# Autodesk Inventor assembly: ENSAMBLAJE_VENTOSA_1
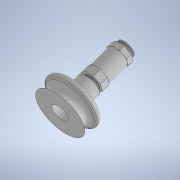
[picture p0: Inventor's stored thumbnail of the model, 180x180]
Saved by Autodesk Inventor 2022 (Build 260153000, 153)
## iProperties
Created: 2022-10-31
Part Number: ENSAMBLAJE_VENTOSA_1
Document SubType Name: Assembly
Designer: Usuario
Author: Usuario
## Documents named in this file (4)
- C:\Users\Usuario\Documents\Cosas de Sebastian\Robotica\PROYECTO\CAD\HERRAMIENTA\ENSAMBLAJE_VENTOSA_1.iam
- C:\Users\Usuario\Documents\Cosas de Sebastian\Robotica\PROYECTO\CAD\HERRAMIENTA\TORNILLO.ipt
- C:\Users\Usuario\Documents\Cosas de Sebastian\Robotica\PROYECTO\CAD\HERRAMIENTA\TUBO_METALICO.ipt
- C:\Users\Usuario\Documents\Cosas de Sebastian\Robotica\PROYECTO\CAD\HERRAMIENTA\VENTOSA.ipt
## Components (3 placed, 3 different names)
1. TORNILLO:1
2. TUBO_METALICO:1
3. VENTOSA:1
## Relationships (3: RevoluteJoint 1, Insert 1, Mate 1)
- [RevoluteJoint]: TORNILLO:1 ↔ VENTOSA:1
- [Insert] (-21 mm): TORNILLO:1 ↔ TUBO_METALICO:1
- [Mate]: TORNILLO:1 ↔ VENTOSA:1
